# Autodesk Inventor assembly: Assembly1
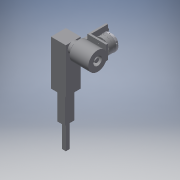
[picture p0: Inventor's stored thumbnail of the model, 180x180]
Saved by Autodesk Inventor 2019 (Build 230136000, 136)
## iProperties
Created: 2020-01-23
Part Number: Assembly1
Document SubType Name: Assembly
Designer: pengj5
Author: pengj5
## Documents named in this file (8)
- C:\Users\Pengj5\OneDrive - Queensland University of Technology\Documents\bracket\NewBracketOrthogonal\NewBracketOrthogonal.iam
- C:\Users\Pengj5\OneDrive - Queensland University of Technology\Documents\bracket\NewBracketOrthogonal\100mm_roller.ipt
- C:\Users\Pengj5\OneDrive - Queensland University of Technology\Documents\bracket\NewBracketOrthogonal\Part1.ipt
- C:\Users\Pengj5\OneDrive - Queensland University of Technology\Documents\bracket\NewBracketOrthogonal\Part2.ipt
- C:\Users\Pengj5\OneDrive - Queensland University of Technology\Documents\bracket\NewBracketOrthogonal\simp_burnisher.ipt
- C:\Users\Pengj5\OneDrive - Queensland University of Technology\Documents\bracket\NewBracketOrthogonal\ATI_9105-IP-2191.ipt
- C:\Users\Pengj5\OneDrive - Queensland University of Technology\Documents\bracket\NewBracketOrthogonal\ATI-3700-05-2126.ipt
- C:\Users\Pengj5\OneDrive - Queensland University of Technology\Documents\bracket\NewBracketOrthogonal\ATI-9105-ECAT-Axia80.ipt
## Components (7 placed, 7 different names)
1. 100mm_roller:1 — Insert:2
2. Part1:1 — Mate:2, Insert:3, Insert:4, Insert:5, Angle:2
3. Part2:1 — Mate:1, Insert:1, Angle:1, Mate:2, Insert:3, Angle:2
4. simp_burnisher:1 — Mate:1, Insert:1, Angle:1, Insert:2
5. ATI_9105-IP-2191:1 — Insert:4, Insert:5, Insert:6
6. ATI-3700-05-2126:1 — Insert:7, Mate:3, Mate:4
7. ATI-9105-ECAT-Axia80:1 — Insert:6, Insert:7
## Relationships (13: Insert 7, Mate 4, Angle 2)
- Mate:1: Part2:1 ↔ simp_burnisher:1
- Insert:1: Part2:1 ↔ simp_burnisher:1
- Angle:1 (0 deg): Part2:1 ↔ simp_burnisher:1
- Insert:2: 100mm_roller:1 ↔ simp_burnisher:1
- Mate:2: Part1:1 ↔ Part2:1
- Insert:3: Part1:1 ↔ Part2:1
- Insert:4: Part1:1 ↔ ATI_9105-IP-2191:1
- Insert:5: Part1:1 ↔ ATI_9105-IP-2191:1
- Insert:6: ATI_9105-IP-2191:1 ↔ ATI-9105-ECAT-Axia80:1
- Insert:7: ATI-3700-05-2126:1 ↔ ATI-9105-ECAT-Axia80:1
- Mate:3: ATI-3700-05-2126:1
- Angle:2 (0 deg): Part1:1 ↔ Part2:1
- Mate:4: ATI-3700-05-2126:1
